# Autodesk Inventor assembly: DriveChain2
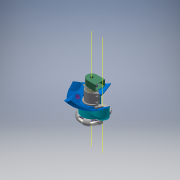
[picture p0: Inventor's stored thumbnail of the model, 180x180]
Saved by Autodesk Inventor 2018.3 (Build 223284000, 284)
## iProperties
Created: 2018-07-27
Part Number: DriveChain2
Material: Generisch
Document SubType Name: Assembly
Designer: JochenAlt
Author: JochenAlt
## Documents named in this file (14)
- D:\Projects\FlowerPot\CAD\DriveChain.iam
- D:\Projects\FlowerPot\CAD\Motor.iam
- D:\Projects\FlowerPot\CAD\HarmonicDrive-Axis.ipt
- D:\Projects\FlowerPot\CAD\BushOmniWheel.ipt
- D:\Projects\FlowerPot\CAD\Mounting Hub.ipt
- D:\Projects\FlowerPot\CAD\Encoder\Avago Encoder.iam
- D:\Projects\FlowerPot\CAD\DriveChainEnclosure2.ipt
- D:\Projects\FlowerPot\CAD\Spindle\SpindleThread.ipt
- D:\Projects\FlowerPot\CAD\Beltdrive\BeltDrive.iam
- D:\Projects\FlowerPot\CAD\AST_Bearings_SMR74ZZ.ipt
- D:\Projects\FlowerPot\CAD\BeltDriveAxis.ipt
- D:\Projects\FlowerPot\CAD\BushBeltDriveTL.ipt
- D:\Projects\FlowerPot\CAD\OmniWheel-70mm-6mm.ipt
- D:\Projects\FlowerPot\CAD\W 637_4 X-2Z.iam
## Components (17 placed, 11 different names)
1. Motor:1 [sub-assembly] — Passend:44, Passend:58, Passend:59, Passend:102
2. HarmonicDrive-Axis:1 — Passend:11, Passend:13, Drehung:4, Passend:82, Drehung:7, Passend:93, Passend:99, Passend:103, Passend:107
3. BushOmniWheel:1 — Passend:11, Passend:14, Passend:109
4. Mounting Hub:1 — Passend:13, Drehung:4, Passend:14, Passend:94, Drehung:8
5. Avago Encoder:1 [sub-assembly] — Passend:58, Passend:59, Winkel:1
6. DriveChainEnclosure:1 — Passend:44, Passend:74, Passend:75, Passend:76, Passend:77, Passend:87, Passend:88, Passend:105, Passend:106
7. SpindleThread:1 — Passend:87, Passend:88
8. BeltDriveTest:1 [sub-assembly] — Drehung:7, Passend:99, Passend:101, Passend:102, Passend:103, Passend:104, Passend:108
9. AST_Bearings_SMR74ZZ:1 — Passend:74, Passend:75, Passend:78, Fluchtend:2, Passend:81
10. AST_Bearings_SMR74ZZ:2 — Passend:76, Passend:77
11. HarmonicDrive-Axis:2 — Passend:78, Fluchtend:2, Passend:79, Passend:80, Passend:85, Passend:104
12. BushOmniWheel:2 — Passend:79
13. BushOmniWheel:3 — Passend:80, Passend:81
14. BushOmniWheel:4 — Passend:82, Passend:101
15. BushOmniWheel:5 — Passend:85
16. OmniWheel:3 — Passend:93, Passend:94, Drehung:8
17. W 637_4 X-2Z:1 [sub-assembly] — Passend:105, Passend:106, Passend:107, Passend:108, Passend:109
## Relationships (35: Mate 30, RelateRotation 3, Flush 1, Angle 1)
- Passend:11 [Mate]: HarmonicDrive-Axis:1 ↔ BushOmniWheel:1
- Passend:13 [Mate]: HarmonicDrive-Axis:1 ↔ Mounting Hub:1
- Drehung:4 [RelateRotation] (1 ul): HarmonicDrive-Axis:1 ↔ Mounting Hub:1
- Passend:14 [Mate]: BushOmniWheel:1 ↔ Mounting Hub:1
- Passend:44 [Mate]: Motor:1 ↔ DriveChainEnclosure:1
- Passend:58 [Mate]: Motor:1 ↔ Avago Encoder:1
- Passend:59 [Mate] (0.5 mm): Motor:1 ↔ Avago Encoder:1
- Passend:74 [Mate]: DriveChainEnclosure:1 ↔ AST_Bearings_SMR74ZZ:1
- Passend:75 [Mate]: DriveChainEnclosure:1 ↔ AST_Bearings_SMR74ZZ:1
- Passend:76 [Mate]: DriveChainEnclosure:1 ↔ AST_Bearings_SMR74ZZ:2
- Passend:77 [Mate]: DriveChainEnclosure:1 ↔ AST_Bearings_SMR74ZZ:2
- Passend:78 [Mate]: AST_Bearings_SMR74ZZ:1 ↔ HarmonicDrive-Axis:2
- Fluchtend:2 [Flush]: AST_Bearings_SMR74ZZ:1 ↔ HarmonicDrive-Axis:2
- Passend:79 [Mate]: HarmonicDrive-Axis:2 ↔ BushOmniWheel:2
- Passend:80 [Mate]: HarmonicDrive-Axis:2 ↔ BushOmniWheel:3
- Passend:81 [Mate]: AST_Bearings_SMR74ZZ:1 ↔ BushOmniWheel:3
- Passend:82 [Mate]: HarmonicDrive-Axis:1 ↔ BushOmniWheel:4
- Passend:85 [Mate]: HarmonicDrive-Axis:2 ↔ BushOmniWheel:5
- Passend:87 [Mate]: DriveChainEnclosure:1 ↔ SpindleThread:1
- Passend:88 [Mate]: DriveChainEnclosure:1 ↔ SpindleThread:1
- Winkel:1 [Angle] (0 deg): Avago Encoder:1
- Drehung:7 [RelateRotation] (1 ul): HarmonicDrive-Axis:1 ↔ BeltDriveTest:1
- Passend:93 [Mate]: HarmonicDrive-Axis:1 ↔ OmniWheel:3
- Passend:94 [Mate]: Mounting Hub:1 ↔ OmniWheel:3
- Passend:99 [Mate]: HarmonicDrive-Axis:1 ↔ BeltDriveTest:1
- Passend:101 [Mate]: BeltDriveTest:1 ↔ BushOmniWheel:4
- Passend:102 [Mate] (0.5 mm): Motor:1 ↔ BeltDriveTest:1
- Passend:103 [Mate]: HarmonicDrive-Axis:1 ↔ BeltDriveTest:1
- Passend:104 [Mate]: BeltDriveTest:1 ↔ HarmonicDrive-Axis:2
- Drehung:8 [RelateRotation] (-1 ul): Mounting Hub:1 ↔ OmniWheel:3
- Passend:105 [Mate]: DriveChainEnclosure:1 ↔ W 637_4 X-2Z:1
- Passend:106 [Mate]: DriveChainEnclosure:1 ↔ W 637_4 X-2Z:1
- Passend:107 [Mate]: HarmonicDrive-Axis:1 ↔ W 637_4 X-2Z:1
- Passend:108 [Mate]: BeltDriveTest:1 ↔ W 637_4 X-2Z:1
- Passend:109 [Mate]: BushOmniWheel:1 ↔ W 637_4 X-2Z:1
